# Autodesk Inventor assembly: Target Holder With Sensors
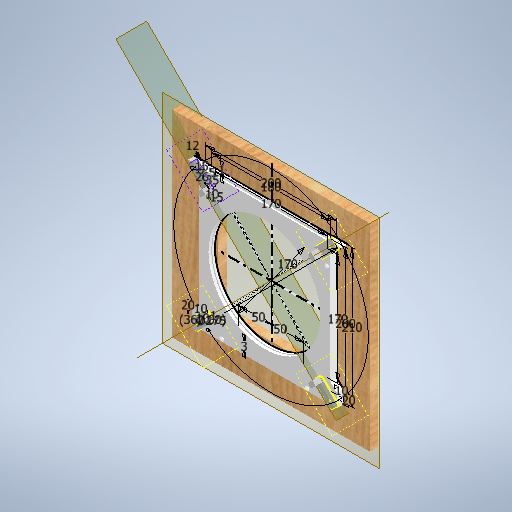
[picture p0: Inventor's stored thumbnail of the model, 512x512]
Saved by Autodesk Inventor 2025.1 (Build 291241000, 241)
## iProperties
Created: 2025-03-25
Part Number: Target Holder With Sensors
Document SubType Name: Assembly
Designer: maxwe
Author: maxwe
## Documents named in this file (7)
- D:\Free E Target\freETarget_wmax\3d Print\Target Holder With Sensors.iam
- D:\Free E Target\freETarget_wmax\3d Print\Front Plate.ipt
- D:\Free E Target\freETarget_wmax\3d Print\Target Holder and Sensor Plate.ipt
- D:\Free E Target\freETarget_wmax\3d Print\Sensor ky-037.ipt
- D:\Free E Target\freETarget_wmax\3d Print\Sensor ky-037_MIR.ipt
- D:\Free E Target\freETarget_wmax\3d Print\Sensor ky-037_MIR1.ipt
- D:\Free E Target\freETarget_wmax\3d Print\Sensor ky-037_MIR_MIR.ipt
## Components (6 placed, 6 different names)
1. Front Plate:1 — Mate:5
2. Target Holder and Sensor Plate:1 — Flush:1, Flush:2, Mate:5, Mate:6, Mate:9, Mate:10, Mate:11
3. Sensor ky-037:1 — Angle:1, Mate:3, Mate:4, Mate:6
4. Sensor ky-037_MIR:1 — Angle:3, Flush:3, Mate:7, Mate:10
5. Sensor ky-037_MIR1:1 — Angle:4, Mate:11, Mate:12, Mate:13
6. Sensor ky-037_MIR_MIR:1 — Mate:8, Mate:9, Flush:4
## Relationships (21: Mate 12, Angle 4, Flush 4, Symmetry 1)
- Angle:1 (-135 deg): Sensor ky-037:1
- Symmetry:1
- Mate:2
- Angle:2 (90 deg)
- Mate:3: Sensor ky-037:1
- Mate:4 (115 mm): Sensor ky-037:1
- Flush:1: Target Holder and Sensor Plate:1
- Flush:2: Target Holder and Sensor Plate:1
- Mate:5: Front Plate:1 ↔ Target Holder and Sensor Plate:1
- Mate:6: Target Holder and Sensor Plate:1 ↔ Sensor ky-037:1
- Angle:3 (-135 deg): Sensor ky-037_MIR:1
- Flush:3 (115 mm): Sensor ky-037_MIR:1
- Angle:4 (-135 deg): Sensor ky-037_MIR1:1
- Mate:7: Sensor ky-037_MIR:1
- Mate:8: Sensor ky-037_MIR_MIR:1
- Mate:9: Target Holder and Sensor Plate:1 ↔ Sensor ky-037_MIR_MIR:1
- Flush:4 (115 mm): Sensor ky-037_MIR_MIR:1
- Mate:10: Target Holder and Sensor Plate:1 ↔ Sensor ky-037_MIR:1
- Mate:11: Target Holder and Sensor Plate:1 ↔ Sensor ky-037_MIR1:1
- Mate:12: Sensor ky-037_MIR1:1
- Mate:13 (115 mm): Sensor ky-037_MIR1:1
